# Autodesk Inventor assembly: Cell stretcher assembly
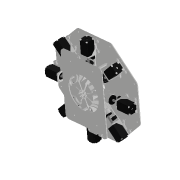
[picture p0: Inventor's stored thumbnail of the model, 180x180]
Saved by Autodesk Inventor 2020 (Build 240168000, 168)
## iProperties
Created: 2022-03-01
Part Number: Cell stretcher assembly
Document SubType Name: Assembly
Designer: ferrerx
Author: ferrerx
## Documents named in this file (5)
- C:\Users\ferrerx\Documents\GitHub\Cell_stretcher_8DOF\Design files\Mechanics\Cell stretcher assembly.iam
- C:\Users\ferrerx\Documents\GitHub\Cell_stretcher_8DOF\Design files\Mechanics\Base.ipt
- C:\Users\ferrerx\Documents\GitHub\Cell_stretcher_8DOF\Design files\Mechanics\Linear actuator.iam
- C:\Users\ferrerx\Documents\GitHub\Cell_stretcher_8DOF\Design files\Mechanics\Microscope lid.ipt
- C:\Users\ferrerx\Documents\GitHub\Cell_stretcher_8DOF\Design files\Mechanics\Electronics spacer.ipt
## Components (12 placed, 4 different names)
1. Base:1 — Mate:1, Mate:2, Mate:3, Mate:10, Mate:11, Mate:12, Mate:13, Mate:14, Mate:15, Mate:16, Mate:17, Mate:18, Mate:19, Mate:20, Mate:21, Mate:22, Mate:23, Mate:24, Mate:25, Mate:26, Mate:27, Mate:28, Mate:29, Mate:30, Mate:51, Mate:52, Mate:53, Mate:54, Mate:55, Mate:56, Mate:57
2. Linear actuator:1 [sub-assembly] — Mate:1, Mate:2, Mate:3
3. Linear actuator:3 [sub-assembly] — Mate:10, Mate:11, Mate:12
4. Linear actuator:4 [sub-assembly] — Mate:13, Mate:14, Mate:15
5. Linear actuator:5 [sub-assembly] — Mate:22, Mate:23, Mate:24
6. Linear actuator:6 [sub-assembly] — Mate:28, Mate:29, Mate:30
7. Linear actuator:7 [sub-assembly] — Mate:16, Mate:17, Mate:18
8. Linear actuator:8 [sub-assembly] — Mate:19, Mate:20, Mate:21
9. Linear actuator:9 [sub-assembly] — Mate:25, Mate:26, Mate:27
10. Microscope lid:1 — Mate:51, Mate:52, Mate:53
11. Electronics spacer:1 — Mate:54, Mate:55
12. Electronics spacer:4 — Mate:56, Mate:57
## Relationships (31: Mate 31)
- Mate:1: Base:1 ↔ Linear actuator:1
- Mate:2: Base:1 ↔ Linear actuator:1
- Mate:3: Base:1 ↔ Linear actuator:1
- Mate:10: Base:1 ↔ Linear actuator:3
- Mate:11: Base:1 ↔ Linear actuator:3
- Mate:12: Base:1 ↔ Linear actuator:3
- Mate:13: Base:1 ↔ Linear actuator:4
- Mate:14: Base:1 ↔ Linear actuator:4
- Mate:15: Base:1 ↔ Linear actuator:4
- Mate:16: Base:1 ↔ Linear actuator:7
- Mate:17: Base:1 ↔ Linear actuator:7
- Mate:18: Base:1 ↔ Linear actuator:7
- Mate:19: Base:1 ↔ Linear actuator:8
- Mate:20: Base:1 ↔ Linear actuator:8
- Mate:21: Base:1 ↔ Linear actuator:8
- Mate:22: Base:1 ↔ Linear actuator:5
- Mate:23: Base:1 ↔ Linear actuator:5
- Mate:24: Base:1 ↔ Linear actuator:5
- Mate:25: Base:1 ↔ Linear actuator:9
- Mate:26: Base:1 ↔ Linear actuator:9
- Mate:27: Base:1 ↔ Linear actuator:9
- Mate:28: Base:1 ↔ Linear actuator:6
- Mate:29: Base:1 ↔ Linear actuator:6
- Mate:30: Base:1 ↔ Linear actuator:6
- Mate:51: Base:1 ↔ Microscope lid:1
- Mate:52: Base:1 ↔ Microscope lid:1
- Mate:53 (30 mm): Base:1 ↔ Microscope lid:1
- Mate:54: Base:1 ↔ Electronics spacer:1
- Mate:55: Base:1 ↔ Electronics spacer:1
- Mate:56: Base:1 ↔ Electronics spacer:4
- Mate:57: Base:1 ↔ Electronics spacer:4
